# Autodesk Inventor assembly: MK3_Assembly
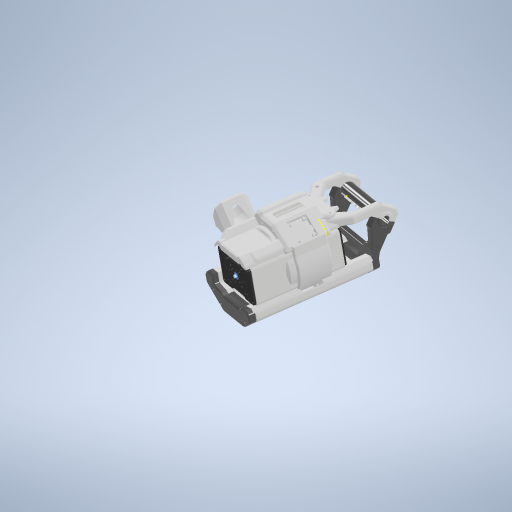
[picture p0: Inventor's stored thumbnail of the model, 512x512]
Saved by Autodesk Inventor 2023.4 (Build 274418000, 418)
## iProperties
Created: 2023-11-16
Part Number: MK3_Assembly
Document SubType Name: Assembly
Designer: aaron
Author: aaron
## Documents named in this file (20)
- C:\work\lunarmass\inventor\r24.01.mk3\MK3_Assembly.iam
- C:\work\lunarmass\inventor\bearings\bearing_58x45x7.ipt
- C:\work\lunarmass\inventor\r23.10.mk3\MotorMountLarge.ipt
- C:\work\lunarmass\inventor\r23.10.mk3\arm_main.ipt
- C:\work\lunarmass\inventor\r24.01.mk3\MK3_DriveTrain.iam
- C:\work\lunarmass\inventor\r24.01.mk3\frame_rring0.ipt
- C:\work\lunarmass\inventor\r24.01.mk3\frame_rring1.ipt
- C:\work\lunarmass\inventor\r24.01.mk3\frame_rring2.ipt
- C:\work\lunarmass\inventor\r24.01.mk3\frame_rring3.ipt
- C:\work\lunarmass\inventor\r24.01.mk3\battery_mnt_left.ipt
- C:\work\lunarmass\inventor\r24.01.mk3\separator_bottom_mid.ipt
- C:\work\lunarmass\inventor\r24.01.mk3\battery_mnt_right.ipt
- C:\work\lunarmass\inventor\r24.01.mk3\bat_cover_left.ipt
- C:\work\lunarmass\inventor\r24.01.mk3\bat_cover_right.ipt
- C:\work\lunarmass\inventor\r24.01.mk3\handle.ipt
- C:\work\lunarmass\inventor\r24.01.mk3\separator_top_mid.ipt
- C:\work\lunarmass\inventor\r24.01.mk3\top_left.ipt
- C:\work\lunarmass\inventor\r24.01.mk3\separator_bottom_mid_cover.ipt
- C:\work\lunarmass\inventor\r24.01.mk3\separator_left.ipt
- C:\work\lunarmass\inventor\r24.01.mk3\temp_holder_mcu.ipt
## Components (20 placed, 19 different names)
1. bearing_58x45x7:1 — Insert:25, Insert:26
2. MotorMountLarge:1 — Insert:22, Insert:23
3. MK3_DriveTrain:1 [sub-assembly] — Insert:18, Insert:19, Insert:26
4. frame_rring0:1 — Insert:18, Insert:19, Insert:20, Flush:1, Mate:5, Mate:8
5. frame_rring1:1 — Insert:20, Insert:33
6. frame_rring2:1 — Insert:21, Mate:1, Insert:25, Mate:4
7. frame_rring3:1 — Insert:21, Mate:1, Insert:22, Insert:23, Mate:2, Mate:3, Flush:1, Mate:11, Mate:12, Mate:13
8. arm_main:1 — Insert:27
9. battery_mnt_left:1 — Mate:2, Mate:3, Mate:4, Insert:27, Insert:29, Insert:30, Mate:15, Mate:16
10. separator_bottom_mid:1 — Mate:7, Flush:2, Mate:15
11. battery_mnt_right:1 — Mate:5, Mate:7, Mate:8, Flush:2, Insert:31, Insert:32, Insert:34
12. bat_cover_left:1 — Insert:29, Insert:30, Mate:10
13. bat_cover_right:1 — Insert:31, Insert:32
14. handle:1 — Flush:3, Mate:9
15. handle:2 — Flush:3, Mate:9, Mate:10
16. separator_top_mid:1 — Insert:33, Mate:11, Mate:14, Insert:35, Flush:4
17. top_left:1 — Mate:12, Mate:13, Mate:14, Mate:17, Flush:5, Flush:6
18. separator_bottom_mid_cover:1 — Insert:34, Mate:16
19. separator_left:1 — Insert:35, Flush:4
20. temp_holder_mcu:1 — Mate:17, Flush:5, Flush:6
## Relationships (38: Insert 16, Mate 16, Flush 6)
- Insert:18: MK3_DriveTrain:1 ↔ frame_rring0:1
- Insert:19: MK3_DriveTrain:1 ↔ frame_rring0:1
- Insert:20: frame_rring0:1 ↔ frame_rring1:1
- Insert:21: frame_rring2:1 ↔ frame_rring3:1
- Mate:1: frame_rring2:1 ↔ frame_rring3:1
- Insert:22: MotorMountLarge:1 ↔ frame_rring3:1
- Insert:23: MotorMountLarge:1 ↔ frame_rring3:1
- Insert:25: bearing_58x45x7:1 ↔ frame_rring2:1
- Insert:26: bearing_58x45x7:1 ↔ MK3_DriveTrain:1
- Mate:2: frame_rring3:1 ↔ battery_mnt_left:1
- Mate:3 (0.05 mm): frame_rring3:1 ↔ battery_mnt_left:1
- Mate:4 (10 mm): frame_rring2:1 ↔ battery_mnt_left:1
- Insert:27 (6 mm): arm_main:1 ↔ battery_mnt_left:1
- Flush:1: frame_rring0:1 ↔ frame_rring3:1
- Mate:5: frame_rring0:1 ↔ battery_mnt_right:1
- Mate:7 (4 mm): separator_bottom_mid:1 ↔ battery_mnt_right:1
- Mate:8 (0.05 mm): frame_rring0:1 ↔ battery_mnt_right:1
- Flush:2: separator_bottom_mid:1 ↔ battery_mnt_right:1
- Insert:29: battery_mnt_left:1 ↔ bat_cover_left:1
- Insert:30: battery_mnt_left:1 ↔ bat_cover_left:1
- Insert:31: battery_mnt_right:1 ↔ bat_cover_right:1
- Insert:32: battery_mnt_right:1 ↔ bat_cover_right:1
- Flush:3: handle:1 ↔ handle:2
- Mate:9: handle:1 ↔ handle:2
- Mate:10: bat_cover_left:1 ↔ handle:2
- Insert:33: frame_rring1:1 ↔ separator_top_mid:1
- Mate:11: frame_rring3:1 ↔ separator_top_mid:1
- Mate:12: frame_rring3:1 ↔ top_left:1
- Mate:13: frame_rring3:1 ↔ top_left:1
- Mate:14: separator_top_mid:1 ↔ top_left:1
- Mate:15: battery_mnt_left:1 ↔ separator_bottom_mid:1
- Insert:34: battery_mnt_right:1 ↔ separator_bottom_mid_cover:1
- Mate:16: battery_mnt_left:1 ↔ separator_bottom_mid_cover:1
- Insert:35: separator_top_mid:1 ↔ separator_left:1
- Flush:4: separator_top_mid:1 ↔ separator_left:1
- Mate:17: top_left:1 ↔ temp_holder_mcu:1
- Flush:5: top_left:1 ↔ temp_holder_mcu:1
- Flush:6 (6 mm): top_left:1 ↔ temp_holder_mcu:1
